# Autodesk Inventor assembly: HingeAssembly
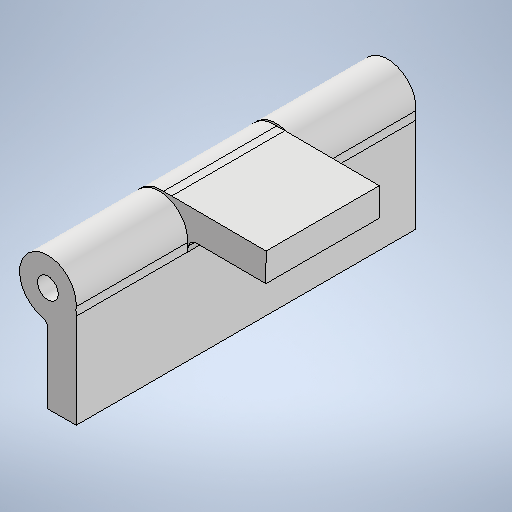
[picture p0: Inventor's stored thumbnail of the model, 512x512]
Saved by Autodesk Inventor 2026 (Build 300175050, 175E)
## iProperties
Created: 2025-10-10
Part Number: HingeAssembly
Document SubType Name: Assembly
Designer: Nicholas M
Author: Nicholas M
## Documents named in this file (3)
- C:\Users\nmari\OneDrive\Documents\Inventor Parts\pinecil-case\Hinge Test\HingeAssembly.iam
- C:\Users\nmari\OneDrive\Documents\Inventor Parts\pinecil-case\Hinge Test\innerhinge.ipt
- C:\Users\nmari\OneDrive\Documents\Inventor Parts\pinecil-case\Hinge Test\outerhinge.ipt
## Components (2 placed, 2 different names)
1. innerhinge:1 — Mate:2, Mate:3
2. outerhinge:1 — Mate:2, Mate:3
## Relationships (2: Mate 2)
- Mate:2: innerhinge:1 ↔ outerhinge:1
- Mate:3 (0.127 mm): innerhinge:1 ↔ outerhinge:1
